# Autodesk Inventor assembly: EG Detector Centellador
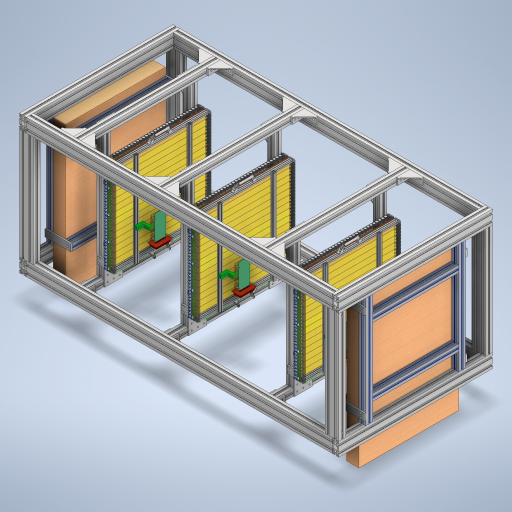
[picture p0: Inventor's stored thumbnail of the model, 512x512]
Saved by Autodesk Inventor 2024.2 (Build 282272000, 272)
## iProperties
Created: 2024-08-29
Part Number: EG Detector Centellador
Document SubType Name: Assembly
Designer: ja.restrepo1
Author: ja.restrepo1
## Documents named in this file (5)
- I:\MICROMECANICA\ALTAS ENERGIAS\Deteccion de Muones\Detectores centelladores\Partes Detector Centellador\EG Detector Centellador.iam
- I:\MICROMECANICA\ALTAS ENERGIAS\Deteccion de Muones\Detectores centelladores\Partes Detector Centellador\SE Chasis DC\SE. Chasis DC.iam
- I:\MICROMECANICA\ALTAS ENERGIAS\Deteccion de Muones\Detectores centelladores\Partes Detector Centellador\SE Chasis DC\SE Chasis Montaje.iam
- I:\MICROMECANICA\ALTAS ENERGIAS\Deteccion de Muones\Detectores centelladores\Partes Detector Centellador\SE cubierta optica\SE cubierta optica.iam
- I:\MICROMECANICA\ALTAS ENERGIAS\Deteccion de Muones\Detectores centelladores\Partes Detector Centellador\SE Base Trigger centellador\SEG soporte Trigger DC.iam
## Components (7 placed, 4 different names)
1. SE. Chasis DC:1 [sub-assembly] — Flush:1, Flush:2, Flush:3, Mate:1, Mate:2, Flush:4, Mate:3, Flush:6, Mate:4, Mate:5, Mate:6, Mate:7, Mate:8, Flush:7, Flush:8, Mate:10, Mate:11, Mate:12
2. SE Chasis Montaje:1 [sub-assembly] — Mate:1, Mate:2, Flush:4, Flush:5
3. SE Chasis Montaje:2 [sub-assembly] — Flush:5, Mate:3
4. SE Chasis Montaje:3 [sub-assembly] — Flush:6, Mate:4
5. SE cubierta optica:1 [sub-assembly] — Mate:5, Mate:6, Mate:7
6. SEG soporte Trigger DC:1 [sub-assembly] — Mate:8, Flush:7, Mate:12
7. SEG soporte Trigger DC:2 [sub-assembly] — Flush:8, Mate:10, Mate:11
## Relationships (19: Mate 11, Flush 8)
- Flush:1: SE. Chasis DC:1
- Flush:2: SE. Chasis DC:1
- Flush:3: SE. Chasis DC:1
- Mate:1: SE. Chasis DC:1 ↔ SE Chasis Montaje:1
- Mate:2: SE. Chasis DC:1 ↔ SE Chasis Montaje:1
- Flush:4: SE. Chasis DC:1 ↔ SE Chasis Montaje:1
- Flush:5: SE Chasis Montaje:1 ↔ SE Chasis Montaje:2
- Mate:3: SE. Chasis DC:1 ↔ SE Chasis Montaje:2
- Flush:6: SE. Chasis DC:1 ↔ SE Chasis Montaje:3
- Mate:4: SE. Chasis DC:1 ↔ SE Chasis Montaje:3
- Mate:5: SE. Chasis DC:1 ↔ SE cubierta optica:1
- Mate:6: SE. Chasis DC:1 ↔ SE cubierta optica:1
- Mate:7: SE. Chasis DC:1 ↔ SE cubierta optica:1
- Mate:8: SE. Chasis DC:1 ↔ SEG soporte Trigger DC:1
- Flush:7: SE. Chasis DC:1 ↔ SEG soporte Trigger DC:1
- Flush:8: SE. Chasis DC:1 ↔ SEG soporte Trigger DC:2
- Mate:10: SE. Chasis DC:1 ↔ SEG soporte Trigger DC:2
- Mate:11 (130 mm): SE. Chasis DC:1 ↔ SEG soporte Trigger DC:2
- Mate:12 (130 mm): SE. Chasis DC:1 ↔ SEG soporte Trigger DC:1
